# Autodesk Inventor assembly: chassis
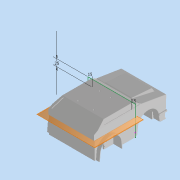
[picture p0: Inventor's stored thumbnail of the model, 180x180]
Saved by Autodesk Inventor 2022 (Build 260153000, 153)
## iProperties
Created: 2021-06-06
Part Number: chassis
Document SubType Name: Assembly
Designer: Default
Author: Default
## Documents named in this file (6)
- E:\source\repos\S21\fachübergreifend\fennec bot\fennec-jet-racer\Konstruktion\chassis.iam
- E:\source\repos\S21\fachübergreifend\fennec bot\fennec-jet-racer\Konstruktion\struktur.ipt
- E:\source\repos\S21\fachübergreifend\fennec bot\fennec-jet-racer\Konstruktion\chassis_front.ipt
- E:\source\repos\S21\fachübergreifend\fennec bot\fennec-jet-racer\Konstruktion\chassis_back_bottomleft.ipt
- E:\source\repos\S21\fachübergreifend\fennec bot\fennec-jet-racer\Konstruktion\chassis_back_bottomright.ipt
- E:\source\repos\S21\fachübergreifend\fennec bot\fennec-jet-racer\Konstruktion\chassis_back_top.ipt
## Components (5 placed, 5 different names)
1. struktur:1 — Passend:1, Passend:2, Passend:3, Passend:4
2. chassis_front:1 — Passend:2, Passend:3, Passend:8, Passend:9
3. chassis_back_bottomleft:1 — Fluchtend:2, Passend:10
4. chassis_back_bottomright:1 — Fluchtend:1, Passend:9, Passend:10
5. chassis_back_top:1 — Passend:8, Fluchtend:1, Fluchtend:2
## Relationships (9: Mate 7, Flush 2)
- Passend:1 [Mate]: struktur:1
- Passend:2 [Mate]: struktur:1 ↔ chassis_front:1
- Passend:3 [Mate]: struktur:1 ↔ chassis_front:1
- Passend:4 [Mate]: struktur:1
- Passend:8 [Mate]: chassis_front:1 ↔ chassis_back_top:1
- Fluchtend:1 [Flush]: chassis_back_bottomright:1 ↔ chassis_back_top:1
- Passend:9 [Mate]: chassis_front:1 ↔ chassis_back_bottomright:1
- Fluchtend:2 [Flush]: chassis_back_bottomleft:1 ↔ chassis_back_top:1
- Passend:10 [Mate]: chassis_back_bottomleft:1 ↔ chassis_back_bottomright:1
